# Autodesk Inventor assembly: ENSAMBLE GENERAL ACH-110L-2021-P
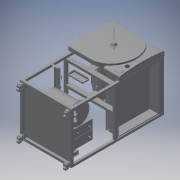
[picture p0: Inventor's stored thumbnail of the model, 180x180]
Saved by Autodesk Inventor 2017 (Build 210142000, 142)
## iProperties
Created: 2021-06-25
Part Number: ENSAMBLE GENERAL ACH-110L-2021-P
Description: STEP AP203
Document SubType Name: Assembly
Designer: USUARIO
Title: ENSAMBLE GENERAL ACH-110L-2021-P.STEP
Revision Number: ANY
Sending System: SolidWorks 2013
Preprocessor: SwSTEP 2.0
## Documents named in this file (33)
- D:\Laboratorio\Autoclave\Autoclave Horizontal\Con Precamara\2021\Autoclave 110L Biocacol OP2021110 #0045886XX\Modelo\ENSAMBLE GENERAL ACH-110L-2021-P.iam
- D:\Laboratorio\Autoclave\Autoclave Horizontal\Con Precamara\2021\Autoclave 110L Biocacol OP2021110 #0045886XX\Modelo\ENSAMBLE CAMARA ACH-110L-2021-P.iam
- D:\Laboratorio\Autoclave\Autoclave Horizontal\Con Precamara\2021\Autoclave 110L Biocacol OP2021110 #0045886XX\Modelo\ESTRUCTURA ACH-110L-2021-P_Predeterminado_Como mecanizada_.ipt
- D:\Laboratorio\Autoclave\Autoclave Horizontal\Con Precamara\2021\Autoclave 110L Biocacol OP2021110 #0045886XX\Modelo\RUEDA SUPO CASTER 250kg.ipt
- D:\Laboratorio\Autoclave\Autoclave Horizontal\Con Precamara\2021\Autoclave 110L Biocacol OP2021110 #0045886XX\Modelo\COMPLEMENTO TUBO ACH-110L-2021-P.ipt
- D:\Laboratorio\Autoclave\Autoclave Horizontal\Con Precamara\2021\Autoclave 110L Biocacol OP2021110 #0045886XX\Modelo\CUBIERTA FRONTAL ACH-110L-2021-P.ipt
- D:\Laboratorio\Autoclave\Autoclave Horizontal\Con Precamara\2021\Autoclave 110L Biocacol OP2021110 #0045886XX\Modelo\ENSAMBLE CUBIERTA POSTERIOR ACH-110L-2021-P.iam
- D:\Laboratorio\Autoclave\Autoclave Horizontal\Con Precamara\2021\Autoclave 110L Biocacol OP2021110 #0045886XX\Modelo\CAJA CONEXIONES ACH-110L-2021-P.ipt
- D:\Laboratorio\Autoclave\Autoclave Horizontal\Con Precamara\2021\Autoclave 110L Biocacol OP2021110 #0045886XX\Modelo\TAPA POSTERIOR ACH-110L-2021-P.ipt
- D:\Laboratorio\Autoclave\Autoclave Horizontal\Con Precamara\2021\Autoclave 110L Biocacol OP2021110 #0045886XX\Modelo\CUBIERTA SUPERIOR ACH-110L-2021-P.ipt
- D:\Laboratorio\Autoclave\Autoclave Horizontal\Con Precamara\2021\Autoclave 110L Biocacol OP2021110 #0045886XX\Modelo\CUBIERTA LATERAL ACH-110L-2021-P.ipt
- D:\Laboratorio\Autoclave\Autoclave Horizontal\Con Precamara\2021\Autoclave 110L Biocacol OP2021110 #0045886XX\Modelo\COMPLEMENTO POSTERIOR ACH-110L-2021-P.ipt
- D:\Laboratorio\Autoclave\Autoclave Horizontal\Con Precamara\2021\Autoclave 110L Biocacol OP2021110 #0045886XX\Modelo\ESPINAS DE PESCADO ACV-ACH.ipt
- D:\Laboratorio\Autoclave\Autoclave Horizontal\Con Precamara\2021\Autoclave 110L Biocacol OP2021110 #0045886XX\Modelo\PG-13,5.ipt
- D:\Laboratorio\Autoclave\Autoclave Horizontal\Con Precamara\2021\Autoclave 110L Biocacol OP2021110 #0045886XX\Modelo\CAJA LUZ DE FONDO ACH-110L-2021-P.ipt
- D:\Laboratorio\Autoclave\Autoclave Horizontal\Con Precamara\2021\Autoclave 110L Biocacol OP2021110 #0045886XX\Modelo\ENSAMBLE CALDERIN ACH-110L-2021-P.iam
- D:\Laboratorio\Autoclave\Autoclave Horizontal\Con Precamara\2021\Autoclave 110L Biocacol OP2021110 #0045886XX\Modelo\ENSAMBLE RESERVORIO BOMBA ACH-110L-2021-P.iam
- D:\Laboratorio\Autoclave\Autoclave Horizontal\Con Precamara\2021\Autoclave 110L Biocacol OP2021110 #0045886XX\Modelo\ENSAMBLE RESERVORIO CALDERIN ACH-110L-2021-P.iam
- D:\Laboratorio\Autoclave\Autoclave Horizontal\Con Precamara\2021\Autoclave 110L Biocacol OP2021110 #0045886XX\Modelo\ENSAMBLE BOMBA DE VACIO VD 27061-2.2.iam
- D:\Laboratorio\Autoclave\Autoclave Horizontal\Con Precamara\2021\Autoclave 110L Biocacol OP2021110 #0045886XX\Modelo\BASE ALUMINIO ACH-110L-2021-P.ipt
- D:\Laboratorio\Autoclave\Autoclave Horizontal\Con Precamara\2021\Autoclave 110L Biocacol OP2021110 #0045886XX\Modelo\SOPORTE VALVULAS ACH-110L-2021-P.ipt
- D:\Laboratorio\Autoclave\Autoclave Horizontal\Con Precamara\2021\Autoclave 110L Biocacol OP2021110 #0045886XX\Modelo\SUJECION VALVULAS ACH-110L-2021-P.ipt
- D:\Laboratorio\Autoclave\Autoclave Horizontal\Con Precamara\2021\Autoclave 110L Biocacol OP2021110 #0045886XX\Modelo\ENSAMBLE PANEL ACH-110L-2021-P.iam
- D:\Laboratorio\Autoclave\Autoclave Horizontal\Con Precamara\2021\Autoclave 110L Biocacol OP2021110 #0045886XX\Modelo\ENSAMBLE PUERTA ACH-110L-2021-P.iam
- D:\Laboratorio\Autoclave\Autoclave Horizontal\Con Precamara\2021\Autoclave 110L Biocacol OP2021110 #0045886XX\Modelo\SOPORTE PUERTA TAPA ACH-110L-2021-P.ipt
- D:\Laboratorio\Autoclave\Autoclave Horizontal\Con Precamara\2021\Autoclave 110L Biocacol OP2021110 #0045886XX\Modelo\IMPRESORA AUTOCLAVE CSN-A2.ipt
- C:\Modelos 3D y DXF\Racores\B122 1-2x1-2.ipt
- C:\Users\USUARIO\Documents\Inventor\Canaleta 40x60 800mm.iam
- C:\Modelos 3D y DXF\Racores\User Library-Tee_Class300.ipt
- C:\Modelos 3D y DXF\Racores\CodoCalle.iam
- C:\Modelos 3D y DXF\Racores\User Library-Valvula-segur-popup-1-2.ipt
- C:\Modelos 3D y DXF\Racores\Check Valve 0.5.ipt
- C:\Modelos 3D y DXF\Danfoss EV210B\DANFOS EV225B.ipt
## Components (42 placed, 40 different names)
1. ENSAMBLE CAMARA ACH-110L-2021-P_1 [sub-assembly] — Insert:1
2. ESTRUCTURA ACH-110L-2021-P_Predeterminado<Como mecanizada>_2
3. RUEDA SUPO CASTER 250kg_3
4. RUEDA SUPO CASTER 250kg_4
5. RUEDA SUPO CASTER 250kg_5
6. RUEDA SUPO CASTER 250kg_6
7. COMPLEMENTO TUBO ACH-110L-2021-P_7
8. COMPLEMENTO TUBO ACH-110L-2021-P_8
9. CUBIERTA FRONTAL ACH-110L-2021-P_9
10. ENSAMBLE CUBIERTA POSTERIOR ACH-110L-2021-P_10 [sub-assembly]
11. CAJA CONEXIONES ACH-110L-2021-P_11 — Mate:1, Flush:1
12. TAPA POSTERIOR ACH-110L-2021-P_12
13. CUBIERTA SUPERIOR ACH-110L-2021-P_13
14. CUBIERTA LATERAL ACH-110L-2021-P_14
15. CUBIERTA LATERAL ACH-110L-2021-P_15
16. COMPLEMENTO POSTERIOR ACH-110L-2021-P_16
17. ESPINAS DE PESCADO ACV-ACH_17
18. PG-13,5_18
19. CAJA LUZ DE FONDO ACH-110L-2021-P_19
20. ENSAMBLE CALDERIN ACH-110L-2021-P_20 [sub-assembly]
21. ENSAMBLE RESERVORIO BOMBA ACH-110L-2021-P_21 [sub-assembly]
22. ENSAMBLE RESERVORIO CALDERIN ACH-110L-2021-P_22 [sub-assembly]
23. ENSAMBLE BOMBA DE VACIO VD 27061-2.2_23 [sub-assembly]
24. BASE ALUMINIO ACH-110L-2021-P_24
25. SOPORTE VALVULAS ACH-110L-2021-P_25
26. SUJECION VALVULAS ACH-110L-2021-P_26
27. SUJECION VALVULAS ACH-110L-2021-P_27
28. SUJECION VALVULAS ACH-110L-2021-P_28
29. SUJECION VALVULAS ACH-110L-2021-P_29
30. ENSAMBLE PANEL ACH-110L-2021-P_30 [sub-assembly]
31. ENSAMBLE PUERTA ACH-110L-2021-P_31 [sub-assembly]
32. SOPORTE PUERTA TAPA ACH-110L-2021-P_32
33. IMPRESORA AUTOCLAVE CSN-A2_33
34. B122 1-2x1-2:1 — Insert:1, Insert:2
35. Canaleta 40x60 800mm:1 [sub-assembly] — Mate:1, Flush:1
36. User Library-Tee_Class300:1 — Insert:2, Insert:3, Insert:5
37. CodoCalle:1 [sub-assembly] — Insert:3, Insert:4
38. User Library-Valvula-segur-popup-1-2:1 — Insert:4
39. B122 1-2x1-2:2 — Insert:5, Insert:6
40. Check Valve 0.5:1 — Insert:6, Insert:7
41. B122 1-2x1-2:3 — Insert:7, Insert:8
42. DANFOS EV225B:1 — Insert:8
## Relationships (10: Insert 8, Mate 1, Flush 1)
- Insert:1 (-9 mm): ENSAMBLE CAMARA ACH-110L-2021-P_1 ↔ B122 1-2x1-2:1
- Mate:1: CAJA CONEXIONES ACH-110L-2021-P_11 ↔ Canaleta 40x60 800mm:1
- Flush:1: CAJA CONEXIONES ACH-110L-2021-P_11 ↔ Canaleta 40x60 800mm:1
- Insert:2 (9 mm): B122 1-2x1-2:1 ↔ User Library-Tee_Class300:1
- Insert:3 (-10 mm): User Library-Tee_Class300:1 ↔ CodoCalle:1
- Insert:4 (-9 mm): CodoCalle:1 ↔ User Library-Valvula-segur-popup-1-2:1
- Insert:5 (-9 mm): User Library-Tee_Class300:1 ↔ B122 1-2x1-2:2
- Insert:6 (-7 mm): B122 1-2x1-2:2 ↔ Check Valve 0.5:1
- Insert:7 (-7 mm): Check Valve 0.5:1 ↔ B122 1-2x1-2:3
- Insert:8 (-9 mm): B122 1-2x1-2:3 ↔ DANFOS EV225B:1
